# Autodesk Inventor assembly: Head
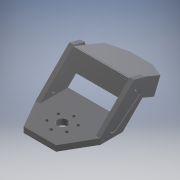
[picture p0: Inventor's stored thumbnail of the model, 180x180]
Saved by Autodesk Inventor 2017 (Build 210142000, 142)
## iProperties
Created: 2018-10-18
Part Number: Head
Document SubType Name: Assembly
Designer: Dell
Author: Dell
## Documents named in this file (11)
- C:\Users\Dell\Documents\GitHub\tr2\Head\Head.iam
- C:\Users\Dell\Documents\GitHub\tr2\Head\HA01.ipt
- C:\Users\Dell\Documents\GitHub\tr2\Head\Orbbec Astra\Orbbec Astra.iam
- C:\Users\Dell\Documents\GitHub\tr2\Head\HA02.ipt
- C:\Users\Dell\Documents\GitHub\tr2\Wheel Assembly\6mm Mounting Hub, thin.ipt
- C:\Users\Dell\Documents\GitHub\tr2\Head\HA03.ipt
- C:\Users\Dell\Documents\GitHub\tr2\Base\37d-gearmotor-50-70-encoder.ipt
- C:\Users\Dell\Documents\GitHub\tr2\Head\HA04.ipt
- C:\Users\Dell\Documents\GitHub\tr2\Head\HA05.ipt
- C:\Users\Dell\Documents\GitHub\tr2\Arm Actuator\Slip Ring.ipt
- C:\Users\Dell\Documents\GitHub\tr2\Head\HA06.ipt
## Components (11 placed, 10 different names)
1. HA01:1 — Mate:11, Mate:12, Mate:13, Mate:14, Mate:16, Mate:17, Mate:29, Mate:30, Angle:1, Mate:31, Mate:32, Mate:33, Mate:34
2. HA02:1 — Mate:4, Mate:21, Mate:22, Mate:23, Mate:24, Mate:25, Mate:26
3. HA03:1 — Mate:11, Mate:12, Mate:13
4. HA04:1 — Mate:21, Mate:22, Mate:23, Mate:36, Mate:38, Mate:39, Mate:40
5. HA05:1 — Mate:24, Mate:25, Mate:26, Mate:27, Mate:29, Mate:35, Mate:41, Mate:42, Mate:43
6. HA06:1 — Mate:38, Mate:39, Mate:40
7. Orbbec Astra:1 [sub-assembly] — Mate:30, Angle:1, Mate:31
8. 37d-gearmotor-50-70-encoder:1 — Mate:14, Mate:16, Mate:17, Mate:19, Mate:35
9. 6mm Mounting Hub, thin:2 — Mate:19, Mate:27
10. Slip Ring:1 — Mate:32, Mate:33, Mate:34, Mate:36
11. HA06:2 — Mate:41, Mate:42, Mate:43
## Relationships (30: Mate 29, Angle 1)
- Mate:4: HA02:1
- Mate:11: HA01:1 ↔ HA03:1
- Mate:12: HA01:1 ↔ HA03:1
- Mate:13: HA01:1 ↔ HA03:1
- Mate:14: HA01:1 ↔ 37d-gearmotor-50-70-encoder:1
- Mate:16: HA01:1 ↔ 37d-gearmotor-50-70-encoder:1
- Mate:17: HA01:1 ↔ 37d-gearmotor-50-70-encoder:1
- Mate:19: 37d-gearmotor-50-70-encoder:1 ↔ 6mm Mounting Hub, thin:2
- Mate:21: HA02:1 ↔ HA04:1
- Mate:22: HA02:1 ↔ HA04:1
- Mate:23: HA02:1 ↔ HA04:1
- Mate:24: HA02:1 ↔ HA05:1
- Mate:25: HA02:1 ↔ HA05:1
- Mate:26: HA02:1 ↔ HA05:1
- Mate:27: HA05:1 ↔ 6mm Mounting Hub, thin:2
- Mate:29: HA01:1 ↔ HA05:1
- Mate:30: HA01:1 ↔ Orbbec Astra:1
- Angle:1 (180 deg): HA01:1 ↔ Orbbec Astra:1
- Mate:31: HA01:1 ↔ Orbbec Astra:1
- Mate:32: HA01:1 ↔ Slip Ring:1
- Mate:33: HA01:1 ↔ Slip Ring:1
- Mate:34: HA01:1 ↔ Slip Ring:1
- Mate:35: HA05:1 ↔ 37d-gearmotor-50-70-encoder:1
- Mate:36: HA04:1 ↔ Slip Ring:1
- Mate:38: HA04:1 ↔ HA06:1
- Mate:39: HA04:1 ↔ HA06:1
- Mate:40: HA04:1 ↔ HA06:1
- Mate:41: HA05:1 ↔ HA06:2
- Mate:42: HA05:1 ↔ HA06:2
- Mate:43: HA05:1 ↔ HA06:2
